# Autodesk Inventor assembly: Lower_Leg_Left
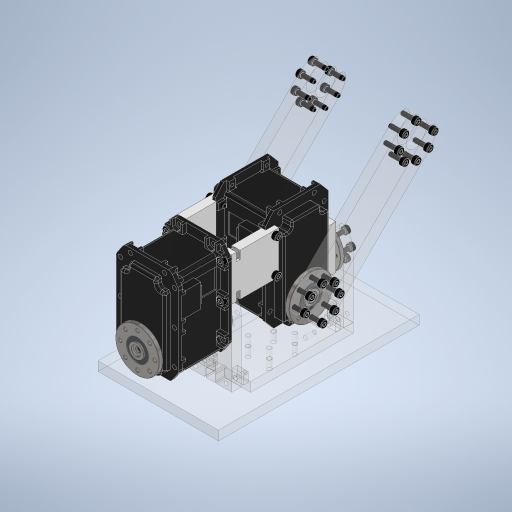
[picture p0: Inventor's stored thumbnail of the model, 512x512]
Saved by Autodesk Inventor 2024 (Build 280153000, 153)
## iProperties
Created: 2024-09-17
Part Number: Lower_Leg_Left
Document SubType Name: Assembly
Designer: Eungang
Author: Eungang
## Documents named in this file (15)
- C:\Users\Eungang\Documents\Inventor\FIGHTING_ROBOT_FINAL\부품\Lower_Leg_Left\Lower_Leg_Left.iam
- C:\Users\Eungang\Documents\Inventor\FIGHTING_ROBOT_FINAL\부품\Lower_Leg_Left\foot_1.ipt
- C:\Users\Eungang\Documents\Inventor\FIGHTING_ROBOT_FINAL\부품\Lower_Leg_Left\foot_2.ipt
- C:\Users\Eungang\Documents\Inventor\FIGHTING_ROBOT_FINAL\부품\Lower_Leg_Left\foot_ankle_bridge.ipt
- C:\Users\Eungang\Documents\Inventor\FIGHTING_ROBOT_FINAL\부품\혼\64-106Horn.ipt
- C:\Users\Eungang\Documents\Inventor\FIGHTING_ROBOT_FINAL\부품\아이들러\64아이들러.iam
- C:\Users\Eungang\Documents\Inventor\FIGHTING_ROBOT_FINAL\부품\Lower_Leg_Left\MX-64T.ipt
- C:\Users\Eungang\Documents\Inventor\FIGHTING_ROBOT_FINAL\부품\Lower_Leg_Left\MX-106T.ipt
- C:\Users\Eungang\Documents\Inventor\FIGHTING_ROBOT_FINAL\부품\Lower_Leg_Left\foot_motor_bridge.ipt
- C:\Users\Eungang\Documents\Inventor\FIGHTING_ROBOT_FINAL\64-106_connect.ipt
- C:\Users\Eungang\Documents\Inventor\FIGHTING_ROBOT_FINAL\부품\Bolt_Washer_Nut\CSH-ST-M2_5-8_203.ipt
- C:\Users\Eungang\Documents\Inventor\FIGHTING_ROBOT_FINAL\부품\Bolt_Washer_Nut\SLBNR2_5.ipt
- C:\Users\Eungang\Documents\Inventor\FIGHTING_ROBOT_FINAL\calf.ipt
- C:\Users\Eungang\Documents\Inventor\FIGHTING_ROBOT_FINAL\부품\Bolt_Washer_Nut\bolt_set_2.5_8 x 7.iam
- C:\Users\Eungang\Documents\Inventor\FIGHTING_ROBOT_FINAL\부품\Lower_Leg_Left\OldVersions\bolt_set_2.5_8 x 7.iam
## Components (47 placed, 13 different names)
1. foot_2:1 — 메이트:2, 삽입:3, 삽입:4, 삽입:5, 삽입:15, 삽입:16
2. foot_ankle_bridge:1 — 삽입:4, 삽입:5, 삽입:10
3. foot_ankle_bridge:2 — 메이트:2, 삽입:3, 삽입:12, 삽입:21, 삽입:47, 삽입:48
4. 64-106Horn:2 — 삽입:10, 삽입:67
5. 64아이들러:2 [sub-assembly] — 삽입:12, 메이트:3, 삽입:21, 메이트:4
6. foot_1:1 — 삽입:15, 삽입:16, 각도:4, 각도:5
7. MX-106T:1 — 삽입:17, 삽입:18, 삽입:19, 삽입:20, 메이트:4, 플러쉬:3, 삽입:53, 삽입:57, 각도:3, 삽입:58, 삽입:59, 삽입:64
8. foot_motor_bridge:1 — 삽입:17, 삽입:18, 메이트:3
9. 64아이들러:3 [sub-assembly] — 삽입:20, 삽입:28, 삽입:32
10. 64-106Horn:3 — 삽입:19, 삽입:27, 삽입:31
11. 64-106_connect:1 — 플러쉬:3, 삽입:53, 삽입:55, 삽입:56
12. CSH-ST-M2_5-8_203:1
13. CSH-ST-M2_5-8_203:3 — 삽입:26
14. SLBNR2_5:2 — 삽입:26
15. calf:7 — 삽입:27, 삽입:31, 삽입:40, 삽입:41, 삽입:42, 삽입:43, 삽입:44, 삽입:45, 삽입:46, 삽입:49, 삽입:50, 각도:4
16. calf:8 — 삽입:28, 삽입:32, 삽입:33, 삽입:34, 삽입:35, 삽입:36, 삽입:37, 삽입:38, 삽입:39, 삽입:51, 삽입:52, 각도:5
17. CSH-ST-M2_5-8_203:4 — 삽입:33
18. CSH-ST-M2_5-8_203:5 — 삽입:34
19. CSH-ST-M2_5-8_203:6 — 삽입:36
20. CSH-ST-M2_5-8_203:7 — 삽입:37
21. CSH-ST-M2_5-8_203:8 — 삽입:35
22. CSH-ST-M2_5-8_203:9 — 삽입:38
23. CSH-ST-M2_5-8_203:10 — 삽입:43
24. CSH-ST-M2_5-8_203:11 — 삽입:42
25. CSH-ST-M2_5-8_203:12 — 삽입:41
26. CSH-ST-M2_5-8_203:13 — 삽입:40
27. CSH-ST-M2_5-8_203:14 — 삽입:44
28. CSH-ST-M2_5-8_203:15 — 삽입:45
29. CSH-ST-M2_5-8_203:22 — 삽입:46
30. CSH-ST-M2_5-8_203:23 — 삽입:39
31. bolt_set_2.5_8 x 7:1 [sub-assembly] — 삽입:47, 삽입:48
32. bolt_set_2.5_8 x 7:2 [sub-assembly] — 삽입:49, 삽입:50
33. bolt_set_2.5_8 x 7:3 [sub-assembly] — 삽입:51, 삽입:52
34. CSH-ST-M2_5-8_203:25
35. SLBNR2_5:3 — 삽입:55
36. CSH-ST-M2_5-8_203:26 — 삽입:56
37. SLBNR2_5:4 — 삽입:57, 각도:3
38. 64-106_connect:2 — 삽입:58, 삽입:59, 삽입:62, 삽입:63, 삽입:65, 삽입:66, 삽입:68
39. CSH-ST-M2_5-8_203:27 — 삽입:63
40. CSH-ST-M2_5-8_203:28 — 삽입:62
41. CSH-ST-M2_5-8_203:29
42. CSH-ST-M2_5-8_203:30
43. SLBNR2_5:5 — 삽입:64
44. SLBNR2_5:6 — 삽입:65
45. SLBNR2_5:7 — 삽입:66
46. 64아이들러:4 [sub-assembly] — 삽입:69
47. MX-64T:1 — 삽입:67, 삽입:68, 삽입:69
## Relationships (58: Insert 51, Mate 3, Angle 3, Flush 1)
- 메이트:2 [Mate] (0.1 mm): foot_2:1 ↔ foot_ankle_bridge:2
- 삽입:3 [Insert]: foot_2:1 ↔ foot_ankle_bridge:2
- 삽입:4 [Insert]: foot_2:1 ↔ foot_ankle_bridge:1
- 삽입:5 [Insert]: foot_2:1 ↔ foot_ankle_bridge:1
- 삽입:10 [Insert]: foot_ankle_bridge:1 ↔ 64-106Horn:2
- 삽입:12 [Insert]: foot_ankle_bridge:2 ↔ 64아이들러:2
- 삽입:15 [Insert]: foot_2:1 ↔ foot_1:1
- 삽입:16 [Insert]: foot_2:1 ↔ foot_1:1
- 삽입:17 [Insert] (0.1 mm): MX-106T:1 ↔ foot_motor_bridge:1
- 삽입:18 [Insert] (0.1 mm): MX-106T:1 ↔ foot_motor_bridge:1
- 메이트:3 [Mate]: 64아이들러:2 ↔ foot_motor_bridge:1
- 삽입:19 [Insert] (0.5 mm): MX-106T:1 ↔ 64-106Horn:3
- 삽입:20 [Insert] (0.5 mm): MX-106T:1 ↔ 64아이들러:3
- 삽입:21 [Insert]: foot_ankle_bridge:2 ↔ 64아이들러:2
- 메이트:4 [Mate]: 64아이들러:2 ↔ MX-106T:1
- 플러쉬:3 [Flush]: MX-106T:1 ↔ 64-106_connect:1
- 삽입:26 [Insert] (0.1 mm): CSH-ST-M2_5-8_203:3 ↔ SLBNR2_5:2
- 삽입:27 [Insert]: 64-106Horn:3 ↔ calf:7
- 삽입:28 [Insert]: 64아이들러:3 ↔ calf:8
- 삽입:31 [Insert]: 64-106Horn:3 ↔ calf:7
- 삽입:32 [Insert]: 64아이들러:3 ↔ calf:8
- 삽입:33 [Insert]: calf:8 ↔ CSH-ST-M2_5-8_203:4
- 삽입:34 [Insert]: calf:8 ↔ CSH-ST-M2_5-8_203:5
- 삽입:35 [Insert]: calf:8 ↔ CSH-ST-M2_5-8_203:8
- 삽입:36 [Insert]: calf:8 ↔ CSH-ST-M2_5-8_203:6
- 삽입:37 [Insert]: calf:8 ↔ CSH-ST-M2_5-8_203:7
- 삽입:38 [Insert]: calf:8 ↔ CSH-ST-M2_5-8_203:9
- 삽입:39 [Insert]: calf:8 ↔ CSH-ST-M2_5-8_203:23
- 삽입:40 [Insert]: calf:7 ↔ CSH-ST-M2_5-8_203:13
- 삽입:41 [Insert]: calf:7 ↔ CSH-ST-M2_5-8_203:12
- 삽입:42 [Insert]: calf:7 ↔ CSH-ST-M2_5-8_203:11
- 삽입:43 [Insert]: calf:7 ↔ CSH-ST-M2_5-8_203:10
- 삽입:44 [Insert]: calf:7 ↔ CSH-ST-M2_5-8_203:14
- 삽입:45 [Insert]: calf:7 ↔ CSH-ST-M2_5-8_203:15
- 삽입:46 [Insert]: calf:7 ↔ CSH-ST-M2_5-8_203:22
- 삽입:47 [Insert]: foot_ankle_bridge:2 ↔ bolt_set_2.5_8 x 7:1
- 삽입:48 [Insert]: foot_ankle_bridge:2 ↔ bolt_set_2.5_8 x 7:1
- 삽입:49 [Insert]: calf:7 ↔ bolt_set_2.5_8 x 7:2
- 삽입:50 [Insert]: calf:7 ↔ bolt_set_2.5_8 x 7:2
- 삽입:51 [Insert]: calf:8 ↔ bolt_set_2.5_8 x 7:3
- 삽입:52 [Insert]: calf:8 ↔ bolt_set_2.5_8 x 7:3
- 삽입:53 [Insert] (0.1 mm): MX-106T:1 ↔ 64-106_connect:1
- 삽입:55 [Insert] (0.1 mm): 64-106_connect:1 ↔ SLBNR2_5:3
- 삽입:56 [Insert]: 64-106_connect:1 ↔ CSH-ST-M2_5-8_203:26
- 삽입:57 [Insert]: MX-106T:1 ↔ SLBNR2_5:4
- 각도:3 [Angle] (0 deg): MX-106T:1 ↔ SLBNR2_5:4
- 삽입:58 [Insert] (0.1 mm): MX-106T:1 ↔ 64-106_connect:2
- 삽입:59 [Insert] (0.1 mm): MX-106T:1 ↔ 64-106_connect:2
- 삽입:62 [Insert]: 64-106_connect:2 ↔ CSH-ST-M2_5-8_203:28
- 삽입:63 [Insert]: 64-106_connect:2 ↔ CSH-ST-M2_5-8_203:27
- 삽입:64 [Insert]: MX-106T:1 ↔ SLBNR2_5:5
- 삽입:65 [Insert] (0.1 mm): 64-106_connect:2 ↔ SLBNR2_5:6
- 삽입:66 [Insert] (0.1 mm): 64-106_connect:2 ↔ SLBNR2_5:7
- 삽입:67 [Insert] (0.5 mm): 64-106Horn:2 ↔ MX-64T:1
- 삽입:68 [Insert]: 64-106_connect:2 ↔ MX-64T:1
- 삽입:69 [Insert] (0.5 mm): 64아이들러:4 ↔ MX-64T:1
- 각도:4 [Angle] (135 deg): foot_1:1 ↔ calf:7
- 각도:5 [Angle] (225 deg): foot_1:1 ↔ calf:8
